# Autodesk Inventor assembly: USBブリッジ基板
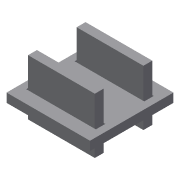
[picture p0: Inventor's stored thumbnail of the model, 180x180]
Saved by Autodesk Inventor 2016 (Build 200138000, 138)
## iProperties
Created: 2016-08-22
Part Number: USBブリッジ基板
Material: 一般
Document SubType Name: Assembly
Designer: NN
Mass: 0.676 g
Surface Area: 11.7268 cm^2
Volume: 0.676 cm^3
Density: 1 g/cm^3
Author: NN
## Documents named in this file (3)
- D:\NN\Dropbox (rt-net)\CAD\RasPiArm\汎用パーツ\USBブリッジ基板\USBブリッジ基板.iam
- D:\NN\Dropbox (rt-net)\CAD\RasPiArm\汎用パーツ\USBブリッジ基板\USBブリッジ基板1.ipt
- D:\NN\Dropbox (rt-net)\CAD\RasPiArm\汎用パーツ\USBブリッジ基板\USBブリッジ基板2.ipt
## Components (3 placed, 2 different names)
1. USBブリッジ基板1:1 — フラッシュ:1, フラッシュ:2
2. USBブリッジ基板2:1 — フラッシュ:2
3. USBブリッジ基板2:2 — フラッシュ:1
## Relationships (2: Flush 2)
- フラッシュ:1 [Flush] (-3 mm): USBブリッジ基板1:1 ↔ USBブリッジ基板2:2
- フラッシュ:2 [Flush] (-3 mm): USBブリッジ基板1:1 ↔ USBブリッジ基板2:1
